# Autodesk Inventor assembly: ASY PNS 2100 cyclone frame
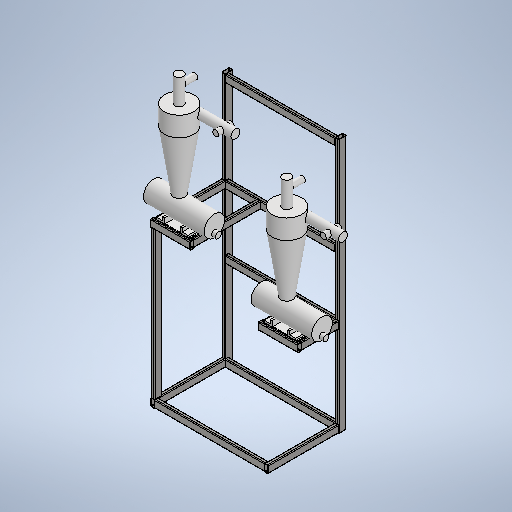
[picture p0: Inventor's stored thumbnail of the model, 512x512]
Saved by Autodesk Inventor 2025.3 (Build 293356030, 356C)
## iProperties
Created: 2025-09-11
Part Number: ASY PNS 2100 cyclone frame
Document SubType Name: Assembly
Designer: admin
Author: admin
## Documents named in this file (4)
- C:\Users\admin\Yandex.Disk\home pc\Inventor\PNS2-Panaevsk\ASY PNS 2100 cyclone frame.iam
- C:\Users\admin\Yandex.Disk\home pc\Inventor\PNS2-Panaevsk\Гидроциклон.ipt
- C:\Users\admin\Yandex.Disk\home pc\Inventor\PNS2-Panaevsk\ASY PNS 2110 cyclone frame.iam
- C:\Users\admin\Yandex.Disk\home pc\Inventor\PNS2-Panaevsk\PNS 2114 cyclone plate.ipt
## Components (5 placed, 3 different names)
1. Гидроциклон:1 — Rigid:3
2. Гидроциклон:2 — Rigid:4
3. ASY PNS 2110 cyclone frame:1 [sub-assembly] — Flush:1, Flush:2, Rigid:1, Rigid:2
4. PNS 2114 cyclone plate:1 — Rigid:1, Rigid:4
5. PNS 2114 cyclone plate:2 — Rigid:2, Rigid:3
## Relationships (6: WeldJoint 4, Flush 2)
- Flush:1: ASY PNS 2110 cyclone frame:1
- Flush:2: ASY PNS 2110 cyclone frame:1
- Rigid:1 [WeldJoint]: ASY PNS 2110 cyclone frame:1 ↔ PNS 2114 cyclone plate:1
- Rigid:2 [WeldJoint]: ASY PNS 2110 cyclone frame:1 ↔ PNS 2114 cyclone plate:2
- Rigid:3 [WeldJoint]: Гидроциклон:1 ↔ PNS 2114 cyclone plate:2
- Rigid:4 [WeldJoint]: Гидроциклон:2 ↔ PNS 2114 cyclone plate:1
